# Autodesk Inventor assembly: wisecoco-assembly
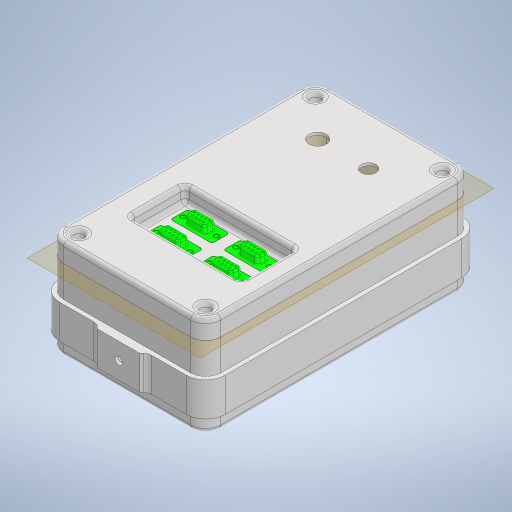
[picture p0: Inventor's stored thumbnail of the model, 512x512]
Saved by Autodesk Inventor 2024 (Build 280153000, 153)
## iProperties
Created: 2024-08-25
Part Number: wisecoco-assembly
Document SubType Name: Assembly
Designer: Stefano
Author: Stefano
## Documents named in this file (10)
- C:\Users\Stefano\Documents\Inventor\Provvedo\inventor-dro-case\wisecoco-version\wisecoco-assembly.iam
- C:\Users\Stefano\Documents\Inventor\Provvedo\inventor-dro-case\wisecoco-version\wisecoco-display.ipt
- C:\Users\Stefano\Documents\Inventor\Provvedo\inventor-dro-case\wisecoco-version\wisecoco-case-body.ipt
- C:\Users\Stefano\Documents\Inventor\Provvedo\inventor-dro-case\wisecoco-version\front-bezel.ipt
- C:\Users\Stefano\Documents\Inventor\Provvedo\inventor-dro-case\wisecoco-version\Rotary Controller V1\Rotary Controller V1.ipt
- C:\Users\Stefano\Documents\Inventor\Provvedo\inventor-dro-case\wisecoco-version\Raspberry Pi 3 .ipt
- C:\Users\Stefano\Documents\Inventor\Provvedo\inventor-dro-case\wisecoco-version\Step\display-retainer-tab.ipt
- C:\Users\Stefano\Documents\Inventor\Provvedo\inventor-dro-case\wisecoco-version\Step\case-back-v2.ipt
- C:\Users\Stefano\Documents\Inventor\Provvedo\inventor-dro-case\Fascia.ipt
- C:\Users\Stefano\Documents\Inventor\Provvedo\inventor-dro-case\wisecoco-version\case-back-v2-connector.ipt
## Components (12 placed, 9 different names)
1. wisecoco-display:1 — Flush:1, Flush:2, Flush:3, Flush:4, Rotational:1, Rotational:2, Mate:4, Mate:5, Mate:6
2. wisecoco-case-body:1 — Flush:1, Flush:2, Flush:5, Flush:8, Flush:11, Flush:12, Cylindrical:1, Cylindrical:8, Rotational:7, Rotational:8
3. front-bezel:1 — Flush:3, Flush:4, Flush:5, Flush:10, Rotational:4, Rotational:5, Rotational:6
4. Rotary Controller V1:1 — Mate:1
5. Raspberry Pi 3 :1 — Rotational:1, Rotational:2, Flush:6
6. display-retainer-tab:1 — Flush:10
7. display-retainer-tab:2 — Rotational:4, Mate:4
8. display-retainer-tab:3 — Rotational:5, Mate:5
9. display-retainer-tab:4 — Rotational:6, Mate:6
10. case-back-v2:1 — Flush:11, Flush:12
11. Fascia:1 — Cylindrical:1, Cylindrical:8
12. case-back-v2-connector:1 — Rotational:7, Rotational:8
## Relationships (23: Flush 10, RevoluteJoint 7, Mate 4, CylindricalJoint 2)
- Flush:1: wisecoco-display:1 ↔ wisecoco-case-body:1
- Flush:2: wisecoco-display:1 ↔ wisecoco-case-body:1
- Flush:3: wisecoco-display:1 ↔ front-bezel:1
- Flush:4 (2.9972 mm): wisecoco-display:1 ↔ front-bezel:1
- Flush:5 (0.508 mm): wisecoco-case-body:1 ↔ front-bezel:1
- Rotational:1 [RevoluteJoint]: wisecoco-display:1 ↔ Raspberry Pi 3 :1
- Rotational:2 [RevoluteJoint]: wisecoco-display:1 ↔ Raspberry Pi 3 :1
- Flush:6 (35 mm): Raspberry Pi 3 :1
- Mate:1: Rotary Controller V1:1
- Flush:8: wisecoco-case-body:1
- Flush:10: front-bezel:1 ↔ display-retainer-tab:1
- Rotational:4 [RevoluteJoint]: front-bezel:1 ↔ display-retainer-tab:2
- Mate:4: wisecoco-display:1 ↔ display-retainer-tab:2
- Rotational:5 [RevoluteJoint]: front-bezel:1 ↔ display-retainer-tab:3
- Rotational:6 [RevoluteJoint]: front-bezel:1 ↔ display-retainer-tab:4
- Mate:5: wisecoco-display:1 ↔ display-retainer-tab:3
- Mate:6: wisecoco-display:1 ↔ display-retainer-tab:4
- Flush:11: wisecoco-case-body:1 ↔ case-back-v2:1
- Flush:12: wisecoco-case-body:1 ↔ case-back-v2:1
- Cylindrical:1: wisecoco-case-body:1 ↔ Fascia:1
- Cylindrical:8: wisecoco-case-body:1 ↔ Fascia:1
- Rotational:7 [RevoluteJoint]: wisecoco-case-body:1 ↔ case-back-v2-connector:1
- Rotational:8 [RevoluteJoint]: wisecoco-case-body:1 ↔ case-back-v2-connector:1
